# Autodesk Inventor assembly: portabateriasConBaterias
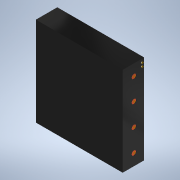
[picture p0: Inventor's stored thumbnail of the model, 180x180]
Saved by Autodesk Inventor 2020 (Build 240168000, 168)
## iProperties
Created: 2022-02-15
Part Number: portabateriasConBaterias
Document SubType Name: Assembly
Designer: DANIEL
Author: DANIEL
## Documents named in this file (3)
- C:\Users\DANIEL\Documents\Personal\Convocatorias\Escollera\tesis\CAD\V3\portabateriasConBaterias.iam
- C:\Users\DANIEL\Documents\Personal\Convocatorias\Escollera\tesis\CAD\V3\portapilas.ipt
- C:\Users\DANIEL\Documents\Personal\Convocatorias\Escollera\tesis\CAD\V3\bateria.ipt
## Components (5 placed, 2 different names)
1. portapilas:1 — Coincidencia:1, Coincidencia:2, Coincidencia:3, Coincidencia:4
2. bateria:1 — Coincidencia:1
3. bateria:2 — Coincidencia:2
4. bateria:3 — Coincidencia:4
5. bateria:4 — Coincidencia:3
## Relationships (4: Mate 4)
- Coincidencia:1 [Mate] (5 mm): portapilas:1 ↔ bateria:1
- Coincidencia:2 [Mate] (5 mm): portapilas:1 ↔ bateria:2
- Coincidencia:3 [Mate] (5 mm): portapilas:1 ↔ bateria:4
- Coincidencia:4 [Mate] (5 mm): portapilas:1 ↔ bateria:3
